# Autodesk Inventor assembly: triangle support
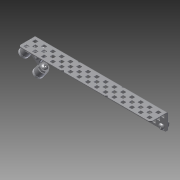
[picture p0: Inventor's stored thumbnail of the model, 180x180]
Saved by Autodesk Inventor 2014 SP1 (Build 180222100, 222)
## iProperties
Created: 2013-09-13
Part Number: triangle support
Document SubType Name: Assembly
Designer: Ryan
Author: Ryan
## Documents named in this file (7)
- C:\Users\Ryan\Desktop\pack and go\Workspaces\Workspace\toss up 1st A bot\toss up tower\triangle support.iam
- C:\Users\Ryan\Desktop\pack and go\Workspaces\Workspace\lib\Aperture VEX CAD Library\Metal\L Bar\2 x 15.ipt
- C:\Users\Ryan\Desktop\pack and go\Workspaces\Workspace\lib\Aperture VEX CAD Library\Bearing Blocks\Pillow Block.ipt
- C:\Users\Ryan\Desktop\pack and go\Workspaces\Workspace\lib\Aperture VEX CAD Library\Hardware\8-32\8-32_.375.ipt
- C:\Users\Ryan\Desktop\pack and go\Workspaces\Workspace\lib\Aperture VEX CAD Library\Spacers\SPACER-0500-0125.ipt
- C:\Users\Ryan\Desktop\pack and go\Workspaces\Workspace\lib\Aperture VEX CAD Library\Spacers\SPACER-0500-0375.ipt
- C:\Users\Ryan\Desktop\pack and go\Workspaces\Workspace\lib\Aperture VEX CAD Library\Hardware\8-32\8-32 nylock.ipt
## Components (12 placed, 6 different names)
1. 2 x 15:1 — Mate:2, Mate:3, Mate:4, Mate:20, Mate:21, Mate:22, Mate:23
2. Pillow Block:1 — Mate:1, Mate:6, Mate:8, Mate:9, Mate:10, Mate:11, Mate:13, Mate:15
3. 8-32_.375:1 — Mate:1, Mate:5, Mate:7
4. SPACER-0500-0125:1 — Mate:2, Mate:3, Mate:4, Mate:5, Mate:6, Mate:7
5. SPACER-0500-0375:1 — Mate:12, Mate:13, Mate:18, Mate:19
6. 8-32_.375:2 — Mate:8, Mate:9, Mate:14
7. 8-32_.375:3 — Mate:10, Mate:11, Mate:12
8. SPACER-0500-0375:2 — Mate:14, Mate:15, Mate:16, Mate:17
9. SPACER-0500-0125:2 — Mate:16, Mate:17
10. SPACER-0500-0125:3 — Mate:18, Mate:19
11. 8-32_.375:4 — Mate:20, Mate:21, Mate:22, Mate:24
12. 8-32 nylock:1 — Mate:23, Mate:24
## Relationships (24: Mate 24)
- Mate:1: Pillow Block:1 ↔ 8-32_.375:1
- Mate:2: 2 x 15:1 ↔ SPACER-0500-0125:1
- Mate:3 (2.3114 mm): 2 x 15:1 ↔ SPACER-0500-0125:1
- Mate:4 (2.3114 mm): 2 x 15:1 ↔ SPACER-0500-0125:1
- Mate:5: 8-32_.375:1 ↔ SPACER-0500-0125:1
- Mate:6 (4.3434 mm): Pillow Block:1 ↔ SPACER-0500-0125:1
- Mate:7 (7.0866 mm): 8-32_.375:1 ↔ SPACER-0500-0125:1
- Mate:8: Pillow Block:1 ↔ 8-32_.375:2
- Mate:9: Pillow Block:1 ↔ 8-32_.375:2
- Mate:10: Pillow Block:1 ↔ 8-32_.375:3
- Mate:11: Pillow Block:1 ↔ 8-32_.375:3
- Mate:12: SPACER-0500-0375:1 ↔ 8-32_.375:3
- Mate:13: Pillow Block:1 ↔ SPACER-0500-0375:1
- Mate:14: 8-32_.375:2 ↔ SPACER-0500-0375:2
- Mate:15: Pillow Block:1 ↔ SPACER-0500-0375:2
- Mate:16: SPACER-0500-0375:2 ↔ SPACER-0500-0125:2
- Mate:17: SPACER-0500-0375:2 ↔ SPACER-0500-0125:2
- Mate:18: SPACER-0500-0375:1 ↔ SPACER-0500-0125:3
- Mate:19: SPACER-0500-0375:1 ↔ SPACER-0500-0125:3
- Mate:20 (2.3114 mm): 2 x 15:1 ↔ 8-32_.375:4
- Mate:21 (1.5875 mm): 2 x 15:1 ↔ 8-32_.375:4
- Mate:22 (2.3114 mm): 2 x 15:1 ↔ 8-32_.375:4
- Mate:23: 2 x 15:1 ↔ 8-32 nylock:1
- Mate:24: 8-32_.375:4 ↔ 8-32 nylock:1
## Named parameters: q = 2.3114 mm
